# Autodesk Inventor assembly: Drone
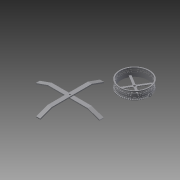
[picture p0: Inventor's stored thumbnail of the model, 180x180]
Saved by Autodesk Inventor 2015 (Build 190159000, 159)
## iProperties
Created: 2015-06-16
Part Number: Drone
Document SubType Name: Assembly
Designer: david_000
Author: david_000
## Documents named in this file (3)
- J:\Drone\Drone.iam
- J:\Drone\Frame.ipt
- J:\Drone\FanChais.iam
## Components (3 placed, 2 different names)
1. Frame:1 — Mate:1, Angle:1, Tangent:1
2. Frame:2 — Mate:1, Angle:1, Tangent:1
3. FanChais:1 [sub-assembly]
## Relationships (3: Mate 1, Angle 1, Tangent 1)
- Mate:1: Frame:1 ↔ Frame:2
- Angle:1 (90 deg): Frame:1 ↔ Frame:2
- Tangent:1: Frame:1 ↔ Frame:2
